# Autodesk Inventor assembly: Carril
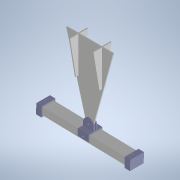
[picture p0: Inventor's stored thumbnail of the model, 180x180]
Saved by Autodesk Inventor 2022 (Build 260153000, 153)
## iProperties
Created: 2022-01-30
Part Number: Carril
Document SubType Name: Assembly
Designer: katha
Author: katha
## Documents named in this file (7)
- C:\Users\katha\OneDrive\Escritorio\Mini_Proyecto_Diseno\Diseno_18012\Modelo_MPD\Carril.iam
- C:\Users\katha\OneDrive\Escritorio\Mini_Proyecto_Diseno\Diseno_18012\Modelo_MPD\Base_Carril.ipt
- C:\Users\katha\OneDrive\Escritorio\Mini_Proyecto_Diseno\Diseno_18012\Modelo_MPD\Lateral_Carril.ipt
- C:\Users\katha\OneDrive\Escritorio\Mini_Proyecto_Diseno\Diseno_18012\Modelo_MPD\Toper_Carril.ipt
- C:\Users\katha\OneDrive\Escritorio\Mini_Proyecto_Diseno\Diseno_18012\Modelo_MPD\Sujetador_Carril.ipt
- C:\Users\katha\OneDrive\Escritorio\Mini_Proyecto_Diseno\Diseno_18012\Modelo_MPD\Pivote_Estructura.ipt
- C:\Users\katha\OneDrive\Escritorio\Mini_Proyecto_Diseno\Diseno_18012\Modelo_MPD\Base_Estructura.ipt
## Components (9 placed, 6 different names)
1. Base_Carril:1 — Flush:1, Mate:1, Mate:2, Mate:3, Mate:4, Mate:5, Mate:6, Mate:7, Mate:8, Mate:9, Mate:10, Mate:11
2. Lateral_Carril:1 — Flush:1, Mate:1, Mate:2
3. Lateral_Carril:2 — Mate:3, Mate:4, Mate:12, Mate:13
4. Toper_Carril:2 — Mate:6, Mate:7, Mate:8
5. Toper_Carril:3 — Mate:5, Mate:9, Mate:10
6. Sujetador_Carril:1 — Mate:11, Mate:12, Mate:13, Mate:14, Mate:15
7. Pivote_Estructura:1 — Flush:2, Mate:14, Mate:15, Mate:16, Mate:17, Mate:18, Mate:19
8. Base_Estructura:1 — Mate:16, Mate:17
9. Base_Estructura:2 — Mate:18, Mate:19
## Relationships (21: Mate 19, Flush 2)
- Flush:1: Base_Carril:1 ↔ Lateral_Carril:1
- Mate:1: Base_Carril:1 ↔ Lateral_Carril:1
- Mate:2: Base_Carril:1 ↔ Lateral_Carril:1
- Mate:3: Base_Carril:1 ↔ Lateral_Carril:2
- Mate:4: Base_Carril:1 ↔ Lateral_Carril:2
- Mate:5: Base_Carril:1 ↔ Toper_Carril:3
- Mate:6: Base_Carril:1 ↔ Toper_Carril:2
- Mate:7: Base_Carril:1 ↔ Toper_Carril:2
- Mate:8 (0.5 mm): Base_Carril:1 ↔ Toper_Carril:2
- Mate:9: Base_Carril:1 ↔ Toper_Carril:3
- Mate:10 (0.5 mm): Base_Carril:1 ↔ Toper_Carril:3
- Mate:11 (0.5 mm): Base_Carril:1 ↔ Sujetador_Carril:1
- Mate:12: Lateral_Carril:2 ↔ Sujetador_Carril:1
- Mate:13 (0.5 mm): Lateral_Carril:2 ↔ Sujetador_Carril:1
- Flush:2: Pivote_Estructura:1
- Mate:14: Sujetador_Carril:1 ↔ Pivote_Estructura:1
- Mate:15 (0.5 mm): Sujetador_Carril:1 ↔ Pivote_Estructura:1
- Mate:16: Pivote_Estructura:1 ↔ Base_Estructura:1
- Mate:17: Pivote_Estructura:1 ↔ Base_Estructura:1
- Mate:18: Pivote_Estructura:1 ↔ Base_Estructura:2
- Mate:19: Pivote_Estructura:1 ↔ Base_Estructura:2
